# Autodesk Inventor assembly: tamiya-slim-tire
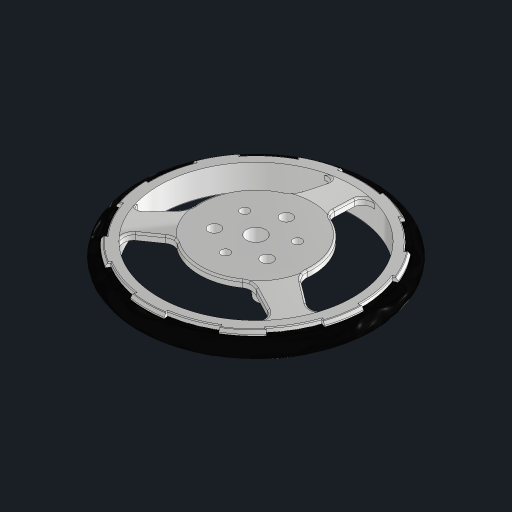
[picture p0: Inventor's stored thumbnail of the model, 512x512]
Saved by Autodesk Inventor 2023.2 (Build 272271030, 271C)
## iProperties
Created: 2023-10-14
Part Number: tamiya-slim-tire
Document SubType Name: Assembly
Designer: takag
Author: takag
## Documents named in this file (3)
- C:\Users\robpl\OneDrive\Documents\Arduino\Onslaught\CAD\tamiya-slim-tire-set-1.snapshot.2\tamiya-slim-tire.iam
- C:\Users\robpl\OneDrive\Documents\Arduino\Onslaught\CAD\tamiya-slim-tire-set-1.snapshot.2\tamiya-slim-tire-wheel.ipt
- C:\Users\robpl\OneDrive\Documents\Arduino\Onslaught\CAD\tamiya-slim-tire-set-1.snapshot.2\tamiya-slim-tire-gomu.ipt
## Components (2 placed, 2 different names)
1. tamiya-slim-tire-wheel:1 — 挿入:1
2. tamiya-slim-tire-gomu:1 — 挿入:1
## Relationships (1: Insert 1)
- 挿入:1 [Insert]: tamiya-slim-tire-wheel:1 ↔ tamiya-slim-tire-gomu:1
